# Autodesk Inventor assembly: new assembly
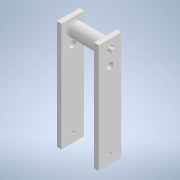
[picture p0: Inventor's stored thumbnail of the model, 180x180]
Saved by Autodesk Inventor 2022 (Build 260153000, 153)
## iProperties
Created: 2022-06-16
Part Number: new assembly
Document SubType Name: Assembly
Designer: chait
Author: chait
## Documents named in this file (5)
- C:\Users\chait\Documents\new assembly.iam
- C:\Users\chait\Documents\Screw 5 mm.ipt
- C:\Users\chait\Documents\spacer.ipt
- C:\Users\chait\Documents\Stationary arm 2.ipt
- C:\Users\chait\Documents\Nylon rod.ipt
## Components (7 placed, 4 different names)
1. Screw 5 mm:1 — Insert:1, Insert:2, Insert:3, Insert:4, Insert:5, Insert:6
2. spacer:1 — Insert:1
3. spacer:2 — Insert:3
4. spacer:3 — Insert:5
5. Stationary arm 2:1 — Insert:2
6. Stationary arm 2:2 — Insert:6
7. Nylon rod:1 — Insert:4
## Relationships (6: Insert 6)
- Insert:1: Screw 5 mm:1 ↔ spacer:1
- Insert:2: Screw 5 mm:1 ↔ Stationary arm 2:1
- Insert:3 (-44 mm): Screw 5 mm:1 ↔ spacer:2
- Insert:4 (-42 mm): Screw 5 mm:1 ↔ Nylon rod:1
- Insert:5 (-10.8 mm): Screw 5 mm:1 ↔ spacer:3
- Insert:6 (-9 mm): Screw 5 mm:1 ↔ Stationary arm 2:2
